# Autodesk Inventor assembly: wahacz_zlozenie
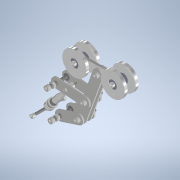
[picture p0: Inventor's stored thumbnail of the model, 180x180]
Saved by Autodesk Inventor 2020.3 (Build 243373000, 373)
## iProperties
Created: 2021-10-24
Part Number: wahacz_zlozenie
Document SubType Name: Assembly
Designer: patry
Author: patry
## Documents named in this file (17)
- C:\Users\patry\Desktop\Konar staff\Ariadna2.1\ariadna_mechanika\Obszar roboczy\Naped\Zawieszenie_v3\wahacz_zlozenie.iam
- C:\Users\patry\Desktop\Konar staff\Ariadna2.1\ariadna_mechanika\Obszar roboczy\Naped\Zawieszenie_v3\glowny_wahacz.ipt
- C:\Users\patry\Desktop\Konar staff\Ariadna2.1\ariadna_mechanika\Obszar roboczy\Naped\Zawieszenie_v3\ramie_1_wahacza.ipt
- C:\Users\patry\Desktop\Konar staff\Ariadna2.1\ariadna_mechanika\Obszar roboczy\Naped\Zawieszenie_v3\ramie_2_wahacza.ipt
- C:\Users\patry\Desktop\Konar staff\Ariadna2.1\ariadna_mechanika\Obszar roboczy\Naped\Zawieszenie_v3\tuleja_TUF106040.ipt
- C:\Users\patry\Desktop\Konar staff\Ariadna2.1\ariadna_mechanika\Obszar roboczy\Naped\Zawieszenie_v3\komplet_kol_V4.iam
- C:\Users\patry\Desktop\Konar staff\Ariadna2.1\ariadna_mechanika\Obszar roboczy\Naped\Sruby\M6_nut_5mm.ipt
- C:\Users\patry\Desktop\Konar staff\Ariadna2.1\ariadna_mechanika\Obszar roboczy\Naped\Sruby\M6x20.ipt
- C:\Users\patry\Desktop\Konar staff\Ariadna2.1\ariadna_mechanika\Obszar roboczy\Naped\Sruby\M6x65.ipt
- C:\Users\patry\Desktop\Konar staff\Ariadna2.1\ariadna_mechanika\Obszar roboczy\Naped\Sruby\M6x35.ipt
- C:\Users\patry\Desktop\Konar staff\Ariadna2.1\ariadna_mechanika\Obszar roboczy\Naped\Amortyzator\Korpus.ipt
- C:\Users\patry\Desktop\Konar staff\Ariadna2.1\ariadna_mechanika\Obszar roboczy\Naped\Amortyzator\Tlok.ipt
- C:\Users\patry\Desktop\Konar staff\Ariadna2.1\ariadna_mechanika\Obszar roboczy\Naped\Amortyzator\Nakretka.ipt
- C:\Users\patry\Desktop\Konar staff\Ariadna2.1\ariadna_mechanika\Obszar roboczy\Naped\Sruby\M3_nut_5mm.ipt
- C:\Users\patry\Desktop\Konar staff\Ariadna2.1\ariadna_mechanika\Obszar roboczy\Naped\Sruby\M3x30.ipt
- C:\Users\patry\Desktop\Konar staff\Ariadna2.1\ariadna_mechanika\Obszar roboczy\Naped\Sruby\M5_nut_5mm.ipt
- C:\Users\patry\Desktop\Konar staff\Ariadna2.1\ariadna_mechanika\Obszar roboczy\Naped\Sruby\M5x65.ipt
## Components (36 placed, 16 different names)
1. glowny_wahacz:1 — Zestawiające:9, Zestawiające:12, Zestawiające:13, Zestawiające:14, Zestawiające:15, Zestawiające:23, Zestawiające:24, Zestawiające:32, Zestawiające:35, Zestawiające:63
2. ramie_1_wahacza:1 — Zestawiające:5, Zestawiające:6, Kątowe:3, Zestawiające:7, Zestawiające:8, Kątowe:4, Zestawiające:39, Zestawiające:51, Zestawiające:74
3. ramie_2_wahacza:1 — Zestawiające:1, Zestawiające:2, Zestawiające:3, Zestawiające:4, Kątowe:1, Kątowe:2, Zestawiające:43, Zestawiające:59
4. tuleja_TUF106040:1 — Zestawiające:1, Zestawiające:2, Kątowe:1, Zestawiające:23, Zestawiające:24, Zestawiające:60
5. tuleja_TUF106040:2 — Zestawiające:3, Zestawiające:4, Kątowe:2, Zestawiające:31
6. tuleja_TUF106040:3 — Zestawiające:5, Zestawiające:6, Kątowe:3, Zestawiające:22, Zestawiające:50
7. tuleja_TUF106040:4 — Zestawiające:7, Zestawiające:8, Kątowe:4, Zestawiające:14, Zestawiające:15
8. komplet_kol_V4:1 [sub-assembly] — Zestawiające:9, Zestawiające:10, Zestawiające:11, Zestawiające:12
9. glowny_wahacz:2 — Zestawiające:10, Zestawiające:11, Zestawiające:13, Zestawiające:20, Zestawiające:21, Zestawiające:29, Zestawiające:30, Zestawiające:33
10. ramie_1_wahacza:2 — Zestawiające:64, Zestawiające:69, Zestawiające:70, Zestawiające:71, Zestawiające:72
11. tuleja_TUF106040:5 — Zestawiające:22
12. tuleja_TUF106040:6 — Zestawiające:20, Zestawiające:21
13. ramie_2_wahacza:2 — Zestawiające:61
14. tuleja_TUF106040:7 — Zestawiające:29, Zestawiające:30
15. tuleja_TUF106040:8 — Zestawiające:31, Zestawiające:58
16. M6_nut_5mm:1 — Zestawiające:34, Zestawiające:35
17. M6x20:1 — Zestawiające:32, Zestawiające:33, Zestawiające:34
18. M6_nut_5mm:2 — Zestawiające:39, Zestawiające:65
19. M6_nut_5mm:3 — Zestawiające:43, Zestawiające:62
20. M6_nut_5mm:4 — Zestawiające:44, Zestawiające:45
21. M6x65:1 — Zestawiające:44, Zestawiające:45, Zestawiające:46, Zestawiające:47, Zestawiające:48, Zestawiające:50
22. M6_nut_5mm:5 — Zestawiające:46, Zestawiające:47, Zestawiające:49
23. M6_nut_5mm:6 — Zestawiające:48, Zestawiające:49, Zestawiające:51
24. M6_nut_5mm:7
25. M6x65:2 — Zestawiające:58, Równoległe:1
26. M6_nut_5mm:8 — Równoległe:2
27. M6_nut_5mm:9 — Zestawiające:59
28. M6x35:1 — Zestawiające:60, Zestawiające:61, Zestawiające:62
29. M6x35:2 — Zestawiające:63, Zestawiające:64, Zestawiające:65
30. Korpus:1 — Zestawiające:75
31. Tlok:1 — Zestawiające:69, Zestawiające:70
32. Nakretka:1
33. M3_nut_5mm:1 — Zestawiające:73, Zestawiające:74
34. M3x30:1 — Zestawiające:71, Zestawiające:72, Zestawiające:73
35. M5_nut_5mm:1 — Zestawiające:76, Równoległe:2
36. M5x65:1 — Zestawiające:75, Zestawiające:76, Równoległe:1
## Relationships (82: Mate 70, Angle 9, Flush 2, CylindricalJoint 1)
- Zestawiające:1 [Mate]: ramie_2_wahacza:1 ↔ tuleja_TUF106040:1
- Zestawiające:2 [Mate]: ramie_2_wahacza:1 ↔ tuleja_TUF106040:1
- Zestawiające:3 [Mate]: ramie_2_wahacza:1 ↔ tuleja_TUF106040:2
- Zestawiające:4 [Mate]: ramie_2_wahacza:1 ↔ tuleja_TUF106040:2
- Kątowe:1 [Angle] (0 deg): ramie_2_wahacza:1 ↔ tuleja_TUF106040:1
- Kątowe:2 [Angle] (0 deg): ramie_2_wahacza:1 ↔ tuleja_TUF106040:2
- Zestawiające:5 [Mate]: ramie_1_wahacza:1 ↔ tuleja_TUF106040:3
- Zestawiające:6 [Mate]: ramie_1_wahacza:1 ↔ tuleja_TUF106040:3
- Kątowe:3 [Angle] (0 deg): ramie_1_wahacza:1 ↔ tuleja_TUF106040:3
- Zestawiające:7 [Mate]: ramie_1_wahacza:1 ↔ tuleja_TUF106040:4
- Zestawiające:8 [Mate]: ramie_1_wahacza:1 ↔ tuleja_TUF106040:4
- Kątowe:4 [Angle] (0 deg): ramie_1_wahacza:1 ↔ tuleja_TUF106040:4
- Zestawiające:9 [Mate]: glowny_wahacz:1 ↔ komplet_kol_V4:1
- Zestawiające:10 [Mate]: komplet_kol_V4:1 ↔ glowny_wahacz:2
- Zestawiające:11 [Mate]: komplet_kol_V4:1 ↔ glowny_wahacz:2
- Zestawiające:12 [Mate]: glowny_wahacz:1 ↔ komplet_kol_V4:1
- Zestawiające:13 [Mate]: glowny_wahacz:1 ↔ glowny_wahacz:2
- Zestawiające:14 [Mate]: glowny_wahacz:1 ↔ tuleja_TUF106040:4
- Zestawiające:15 [Mate] (2.5 mm): glowny_wahacz:1 ↔ tuleja_TUF106040:4
- [Mate]: ramie_1_wahacza:2 ↔ tuleja_TUF106040:5
- [Mate]: ramie_1_wahacza:2 ↔ tuleja_TUF106040:5
- [Angle] (0 deg): ramie_1_wahacza:2 ↔ tuleja_TUF106040:5
- [Mate]: ramie_1_wahacza:2 ↔ tuleja_TUF106040:6
- [Mate]: ramie_1_wahacza:2 ↔ tuleja_TUF106040:6
- [Angle] (0 deg): ramie_1_wahacza:2 ↔ tuleja_TUF106040:6
- Zestawiające:20 [Mate] (2.5 mm): glowny_wahacz:2 ↔ tuleja_TUF106040:6
- Zestawiające:21 [Mate]: glowny_wahacz:2 ↔ tuleja_TUF106040:6
- Zestawiające:22 [Mate]: tuleja_TUF106040:3 ↔ tuleja_TUF106040:5
- Zestawiające:23 [Mate] (2.5 mm): glowny_wahacz:1 ↔ tuleja_TUF106040:1
- Zestawiające:24 [Mate]: glowny_wahacz:1 ↔ tuleja_TUF106040:1
- [Mate]: ramie_2_wahacza:2 ↔ tuleja_TUF106040:7
- [Mate]: ramie_2_wahacza:2 ↔ tuleja_TUF106040:7
- [Mate]: ramie_2_wahacza:2 ↔ tuleja_TUF106040:8
- [Mate]: ramie_2_wahacza:2 ↔ tuleja_TUF106040:8
- [Angle] (0 deg): ramie_2_wahacza:2 ↔ tuleja_TUF106040:7
- [Angle] (0 deg): ramie_2_wahacza:2 ↔ tuleja_TUF106040:8
- Zestawiające:29 [Mate] (2.5 mm): glowny_wahacz:2 ↔ tuleja_TUF106040:7
- Zestawiające:30 [Mate]: glowny_wahacz:2 ↔ tuleja_TUF106040:7
- Zestawiające:31 [Mate]: tuleja_TUF106040:2 ↔ tuleja_TUF106040:8
- Zestawiające:32 [Mate]: glowny_wahacz:1 ↔ M6x20:1
- Zestawiające:33 [Mate]: glowny_wahacz:2 ↔ M6x20:1
- Zestawiające:34 [Mate]: M6_nut_5mm:1 ↔ M6x20:1
- Zestawiające:35 [Mate]: glowny_wahacz:1 ↔ M6_nut_5mm:1
- Zestawiające:39 [Mate]: ramie_1_wahacza:1 ↔ M6_nut_5mm:2
- Zestawiające:43 [Mate]: ramie_2_wahacza:1 ↔ M6_nut_5mm:3
- Zestawiające:44 [Mate]: M6_nut_5mm:4 ↔ M6x65:1
- Zestawiające:45 [Mate] (5 mm): M6_nut_5mm:4 ↔ M6x65:1
- Zestawiające:46 [Mate] (-5 mm): M6x65:1 ↔ M6_nut_5mm:5
- Zestawiające:47 [Mate]: M6x65:1 ↔ M6_nut_5mm:5
- Zestawiające:48 [Mate]: M6x65:1 ↔ M6_nut_5mm:6
- Zestawiające:49 [Mate] (5 mm): M6_nut_5mm:5 ↔ M6_nut_5mm:6
- Zestawiające:50 [Mate]: tuleja_TUF106040:3 ↔ M6x65:1
- Zestawiające:51 [Mate] (9.5 mm): ramie_1_wahacza:1 ↔ M6_nut_5mm:6
- [Mate]: M6_nut_5mm:7 ↔ M6x65:2
- [Mate] (5 mm): M6_nut_5mm:7 ↔ M6x65:2
- [Mate] (-5 mm): M6x65:2 ↔ M6_nut_5mm:8
- [Mate]: M6x65:2 ↔ M6_nut_5mm:8
- [Mate]: M6x65:2 ↔ M6_nut_5mm:9
- [Mate] (5 mm): M6_nut_5mm:8 ↔ M6_nut_5mm:9
- Zestawiające:58 [Mate]: tuleja_TUF106040:8 ↔ M6x65:2
- Zestawiające:59 [Mate] (9.5 mm): ramie_2_wahacza:1 ↔ M6_nut_5mm:9
- Zestawiające:60 [Mate]: tuleja_TUF106040:1 ↔ M6x35:1
- Zestawiające:61 [Mate]: ramie_2_wahacza:2 ↔ M6x35:1
- Zestawiające:62 [Mate]: M6_nut_5mm:3 ↔ M6x35:1
- Zestawiające:63 [Mate]: glowny_wahacz:1 ↔ M6x35:2
- Zestawiające:64 [Mate]: ramie_1_wahacza:2 ↔ M6x35:2
- Zestawiające:65 [Mate]: M6_nut_5mm:2 ↔ M6x35:2
- [Mate]: Korpus:1 ↔ Tlok:1
- [Angle] (0 deg): Korpus:1 ↔ Tlok:1
- [Mate]: Korpus:1 ↔ Nakretka:1
- [Mate] (5 mm): Korpus:1 ↔ Nakretka:1
- [CylindricalJoint]: Korpus:1 ↔ Tlok:1
- Zestawiające:69 [Mate]: ramie_1_wahacza:2 ↔ Tlok:1
- Zestawiające:70 [Mate] (7.5 mm): ramie_1_wahacza:2 ↔ Tlok:1
- Zestawiające:71 [Mate]: ramie_1_wahacza:2 ↔ M3x30:1
- Zestawiające:72 [Mate]: ramie_1_wahacza:2 ↔ M3x30:1
- Zestawiające:73 [Mate]: M3_nut_5mm:1 ↔ M3x30:1
- Zestawiające:74 [Mate]: ramie_1_wahacza:1 ↔ M3_nut_5mm:1
- Zestawiające:75 [Mate]: Korpus:1 ↔ M5x65:1
- Zestawiające:76 [Mate]: M5_nut_5mm:1 ↔ M5x65:1
- Równoległe:1 [Flush]: M6x65:2 ↔ M5x65:1
- Równoległe:2 [Flush]: M6_nut_5mm:8 ↔ M5_nut_5mm:1
## Named parameters: d29_d6 = 0 mm, d30_d7 = 0 mm, d31_d8 = 0 deg, d32_d9 = 0 mm, d33_d10 = 0 mm, d34_d11 = 0 deg, d40_d3 = 0 mm, d41_d4 = 0 deg, d42_d5 = 0 deg, d43_d0 = 0 mm, d44_d1 = 0 mm, d45_d2 = 0 mm, d69_d66 = 5 mm, d70_d61 = 0 mm, d71_d62 = 5 mm, d72_d63 = -5 mm, d73_d64 = 0 mm, d74_d65 = 0 mm, d83_d6 = -2 mm, d84_d7 = -1.99993 mm, d85_d8 = -15 mm, d86_d0 = 0 mm, d87_d1 = 0 deg, d88_d3 = 0 mm, d89_d4 = 5 mm, d90_d5 = 0 deg
